# Autodesk Inventor assembly: Slider_crank_mechanism
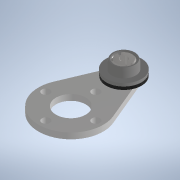
[picture p0: Inventor's stored thumbnail of the model, 180x180]
Saved by Autodesk Inventor 2020.4 (Build 244396000, 396)
## iProperties
Created: 2021-09-06
Part Number: Slider_crank_mechanism
Document SubType Name: Assembly
Designer: Masato
Mass: 2.53036 g
Surface Area: 18.5815 cm^2
Volume: 1.13409 cm^3
Density: 2.23118 g/cm^3
Author: Masato
## Documents named in this file (5)
- C:\Users\Masato\Documents\Inventor\CIT Brains_Inventor\名称変更\OpenPlatform_ver3_0\LowerBody\長穴減速\Slider_crank_mechanism.iam
- C:\Users\Masato\Documents\Inventor\CIT Brains_Inventor\名称変更\OpenPlatform_ver3_0\LowerBody\長穴減速\Slider_crank_horn.ipt
- C:\Users\Masato\Documents\Inventor\CIT Brains_Inventor\名称変更\OpenPlatform_ver3_0\Ready_Made\80F-0603.ipt
- C:\Users\Masato\Documents\Inventor\CIT Brains_Inventor\名称変更\OpenPlatform_ver3_0\Ready_Made\ARU-304S.ipt
- C:\Users\Masato\Documents\Inventor\CIT Brains_Inventor\名称変更\OpenPlatform_ver3_0\Ready_Made\UUW-0312-10BH.ipt
## Components (4 placed, 4 different names)
1. Slider_crank_horn:1 — 挿入:1
2. 80F-0603:1 — 挿入:2
3. ARU-304S:1 — 挿入:3
4. UUW-0312-10BH:1 — 挿入:1, 挿入:2, 挿入:3
## Relationships (3: Insert 3)
- 挿入:1 [Insert]: Slider_crank_horn:1 ↔ UUW-0312-10BH:1
- 挿入:2 [Insert]: 80F-0603:1 ↔ UUW-0312-10BH:1
- 挿入:3 [Insert]: ARU-304S:1 ↔ UUW-0312-10BH:1
